# Autodesk Inventor assembly: TailwAilerons
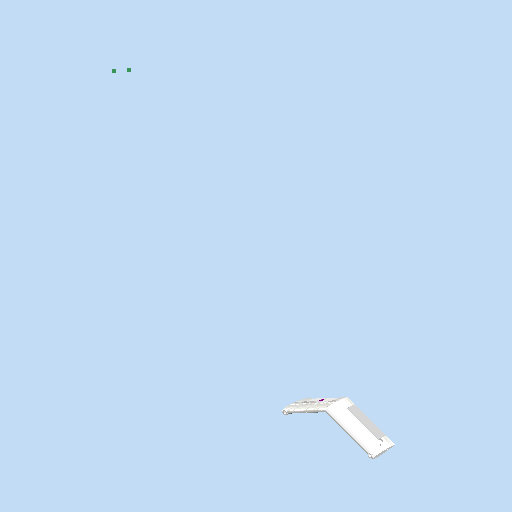
[picture p0: Inventor's stored thumbnail of the model, 512x512]
Saved by Autodesk Inventor 2026.1 (Build 301233000, 233)
## iProperties
Created: 2026-03-18
Part Number: TailwAilerons
Document SubType Name: Assembly
Designer: mateo
Author: mateo
## Documents named in this file (4)
- C:\GitHub\Senior-Design-UAV\Elytra CAD\Assembly\TailwAilerons.iam
- C:\GitHub\Senior-Design-UAV\Elytra CAD\Tail.ipt
- C:\GitHub\Senior-Design-UAV\Elytra CAD\Ailerons\VTailAilerons.ipt
- C:\GitHub\Senior-Design-UAV\Elytra CAD\Ailerons\Vtail_MIR.ipt
## Components (3 placed, 3 different names)
1. Tail:1 — Mate:1, Mate:2
2. VTailAilerons:1 — Mate:1
3. Vtail_MIR:1 — Mate:2
## Relationships (2: Mate 2)
- Mate:1 (0.125 mm): Tail:1 ↔ VTailAilerons:1
- Mate:2 (0.125 mm): Tail:1 ↔ Vtail_MIR:1
